# Autodesk Inventor assembly: !tower
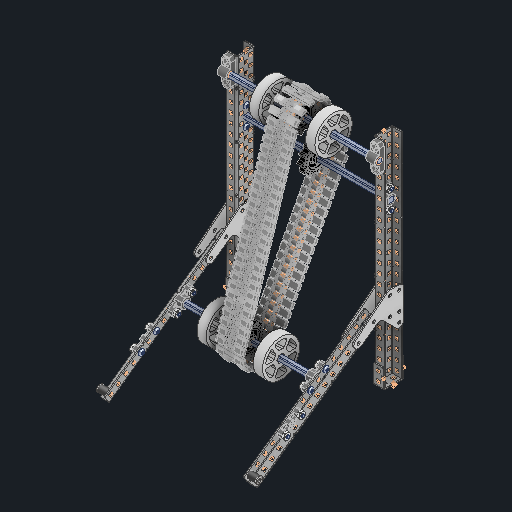
[picture p0: Inventor's stored thumbnail of the model, 512x512]
Saved by Autodesk Inventor 2025 (Build 290162000, 162)
## iProperties
Created: 2024-10-13
Part Number: !tower
Document SubType Name: Assembly
Designer: Averey Ku
Author: Averey Ku
## Documents named in this file (12)
- D:\vex_robotics_high_stakes\hardware\cad\bots\high_stakes_v2\tower\!tower.iam
- D:\vex_robotics_high_stakes\hardware\cad\bots\high_stakes_v2\tower\structure\!structure.iam
- D:\vex_robotics_high_stakes\hardware\cad\robpros_cad_lib\Motion\Shaft HS\Shaft HS\Shaft HS 7.5 in.ipt
- D:\vex_robotics_high_stakes\hardware\cad\robpros_cad_lib\Motion\Shaft HS\Shaft HS.ipt
- D:\vex_robotics_high_stakes\hardware\cad\robpros_cad_lib\Motion\Sprockets\9P Sprocket.iam
- D:\vex_robotics_high_stakes\hardware\cad\robpros_cad_lib\Motion\Sprockets\9P Sprocket\9P 12T Sprocket, No Insert.iam
- D:\vex_robotics_high_stakes\hardware\cad\robpros_cad_lib\Motion\Wheels\Flex Wheels\2.000 Flex Wheel\2.000 30A .500.ipt
- D:\vex_robotics_high_stakes\hardware\cad\robpros_cad_lib\Motion\Wheels\Flex Wheels\2.000 Flex Wheel.ipt
- D:\vex_robotics_high_stakes\hardware\cad\robpros_cad_lib\Motion\Shaft HS\Shaft HS\Shaft HS 8.5 in.ipt
- D:\vex_robotics_high_stakes\hardware\cad\bots\high_stakes_v2\tower\chain_path.ipt
- D:\vex_robotics_high_stakes\hardware\cad\robpros_cad_lib\Motion\Chain 9P\Tank Tread Traction Link.ipt
- D:\vex_robotics_high_stakes\hardware\cad\robpros_cad_lib\Motion\Chain 9P\Chain Attachment Link.ipt
## Components (76 placed, 8 different names)
1. !structure:1 [sub-assembly] — Insert:1, Insert:2, Insert:5, Insert:8
2. Shaft HS 7.5 in:1 — Insert:1
3. 9P 12T Sprocket, No Insert:2 [sub-assembly] — Insert:2, Insert:3, Insert:4, Flush:1, Flush:3
4. 2.000 30A .500:1 — Insert:3
5. 2.000 30A .500:2 — Insert:4
6. Shaft HS 8.5 in:2 — Insert:5, Mate:1
7. 9P 12T Sprocket, No Insert:3 [sub-assembly] — Flush:1, Mate:1, Insert:6, Insert:7, Flush:2, Mate:3
8. 2.000 30A .500:3 — Insert:6
9. 2.000 30A .500:4 — Insert:7
10. Shaft HS 8.5 in:3 — Insert:8, Mate:2
11. 9P 12T Sprocket, No Insert:4 [sub-assembly] — Flush:2, Mate:2
12. chain_path:1 — Flush:3, Mate:4, Angle:1
13. Chain Attachment Link:1 — Insert:9, Mate:5
14. Tank Tread Traction Link:1 — Mate:3, Mate:4, Angle:1
15. Tank Tread Traction Link:2
16. Tank Tread Traction Link:3
17. Tank Tread Traction Link:4
18. Tank Tread Traction Link:5
19. Tank Tread Traction Link:6
20. Tank Tread Traction Link:7
21. Tank Tread Traction Link:8
22. Tank Tread Traction Link:9
23. Tank Tread Traction Link:10
24. Tank Tread Traction Link:11
25. Tank Tread Traction Link:12
26. Tank Tread Traction Link:13
27. Tank Tread Traction Link:14
28. Tank Tread Traction Link:15
29. Tank Tread Traction Link:16
30. Tank Tread Traction Link:17
31. Tank Tread Traction Link:18
32. Tank Tread Traction Link:19
33. Tank Tread Traction Link:20
34. Tank Tread Traction Link:21
35. Tank Tread Traction Link:22
36. Tank Tread Traction Link:23
37. Tank Tread Traction Link:24
38. Tank Tread Traction Link:25
39. Tank Tread Traction Link:26
40. Tank Tread Traction Link:27
41. Tank Tread Traction Link:28
42. Tank Tread Traction Link:29
43. Tank Tread Traction Link:30
44. Tank Tread Traction Link:31
45. Tank Tread Traction Link:32
46. Tank Tread Traction Link:33
47. Tank Tread Traction Link:34
48. Tank Tread Traction Link:35
49. Tank Tread Traction Link:36
50. Tank Tread Traction Link:37
51. Tank Tread Traction Link:38
52. Tank Tread Traction Link:39
53. Tank Tread Traction Link:40
54. Tank Tread Traction Link:41
55. Tank Tread Traction Link:42
56. Tank Tread Traction Link:43
57. Tank Tread Traction Link:44
58. Tank Tread Traction Link:45
59. Tank Tread Traction Link:46
60. Tank Tread Traction Link:47
61. Tank Tread Traction Link:48
62. Tank Tread Traction Link:49
63. Tank Tread Traction Link:50
64. Tank Tread Traction Link:51
65. Tank Tread Traction Link:52
66. Tank Tread Traction Link:53 — Insert:9, Mate:5
67. Tank Tread Traction Link:54
68. Tank Tread Traction Link:55
69. Tank Tread Traction Link:56
70. Tank Tread Traction Link:57
71. Tank Tread Traction Link:58
72. Tank Tread Traction Link:59
73. Tank Tread Traction Link:60
74. Tank Tread Traction Link:61
75. Tank Tread Traction Link:62
76. Tank Tread Traction Link:63
## Component patterns: (63 elements, first: Tank Tread Traction Link:1)
## Relationships (18: Insert 9, Mate 5, Flush 3, Angle 1)
- Insert:1: !structure:1 ↔ Shaft HS 7.5 in:1
- Insert:2 (87.9094 mm): !structure:1 ↔ 9P 12T Sprocket, No Insert:2
- Insert:3 (25.4 mm): 9P 12T Sprocket, No Insert:2 ↔ 2.000 30A .500:1
- Insert:4 (25.4 mm): 9P 12T Sprocket, No Insert:2 ↔ 2.000 30A .500:2
- Insert:5: !structure:1 ↔ Shaft HS 8.5 in:2
- Flush:1: 9P 12T Sprocket, No Insert:2 ↔ 9P 12T Sprocket, No Insert:3
- Mate:1: Shaft HS 8.5 in:2 ↔ 9P 12T Sprocket, No Insert:3
- Insert:6 (25.4 mm): 9P 12T Sprocket, No Insert:3 ↔ 2.000 30A .500:3
- Insert:7 (25.4 mm): 9P 12T Sprocket, No Insert:3 ↔ 2.000 30A .500:4
- Insert:8: !structure:1 ↔ Shaft HS 8.5 in:3
- Flush:2: 9P 12T Sprocket, No Insert:3 ↔ 9P 12T Sprocket, No Insert:4
- Mate:2: Shaft HS 8.5 in:3 ↔ 9P 12T Sprocket, No Insert:4
- Flush:3: 9P 12T Sprocket, No Insert:2 ↔ chain_path:1
- Mate:3: 9P 12T Sprocket, No Insert:3 ↔ Tank Tread Traction Link:1
- Mate:4: chain_path:1 ↔ Tank Tread Traction Link:1
- Angle:1 (-90 deg): chain_path:1 ↔ Tank Tread Traction Link:1
- Insert:9: Chain Attachment Link:1 ↔ Tank Tread Traction Link:53
- Mate:5: Chain Attachment Link:1 ↔ Tank Tread Traction Link:53
